# Autodesk Inventor assembly: 1420-06-00 Endstop
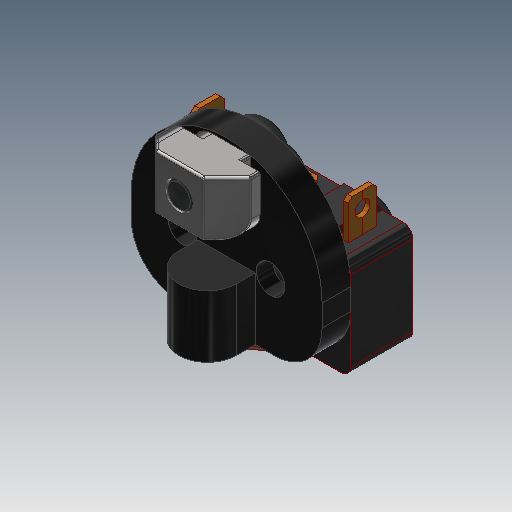
[picture p0: Inventor's stored thumbnail of the model, 512x512]
Saved by Autodesk Inventor 2017 (Build 210142000, 142)
## iProperties
Part Number: 1420-06-00 Endstop
Material: Générique
Document SubType Name: Assembly
Designer: Adrien MARY
Author: Adrien MARY
## Documents named in this file (5)
- W:\Professionnel\Conception FABLAB\1420-Vauban 3D XL\1420-06 Endstop\1420-06-00 Endstop.iam
- W:\Professionnel\Conception FABLAB\1420-Vauban 3D XL\1420-06 Endstop\1420-06-01 Support capteur.ipt
- W:\Professionnel\Conception FABLAB\1420-Vauban 3D XL\1420-06 Endstop\1420-06-02 Endstop.ipt
- W:\Professionnel\Conception FABLAB\1420-Vauban 3D XL\1420-90 Centre de contenu\fr-FR\ISO 7380-1\ISO 7380-1 - M3 x 8.ipt
- W:\Professionnel\Conception FABLAB\1420-Vauban 3D XL\1420-01 Armature\1420-01-11 Noix M3.ipt
## Components (6 placed, 4 different names)
1. 1420-06-01 Support capteur:1 — Logement:1, Placage:1, Logement:4, Affleurement:1
2. 1420-06-02 Endstop:1 — Logement:1, Placage:1, Logement:2, Logement:3
3. ISO 7380-1 M3 x 8:1 — Logement:3
4. ISO 7380-1 M3 x 8:2 — Logement:2
5. ISO 7380-1 M3 x 8:3 — Logement:4, Placage:2
6. 1420-01-11 Noix M3:1 — Affleurement:1, Placage:2
## Relationships (7: Insert 4, Mate 2, Flush 1)
- Logement:1 [Insert]: 1420-06-01 Support capteur:1 ↔ 1420-06-02 Endstop:1
- Placage:1 [Mate]: 1420-06-01 Support capteur:1 ↔ 1420-06-02 Endstop:1
- Logement:2 [Insert]: 1420-06-02 Endstop:1 ↔ ISO 7380-1 M3 x 8:2
- Logement:3 [Insert]: 1420-06-02 Endstop:1 ↔ ISO 7380-1 M3 x 8:1
- Logement:4 [Insert]: 1420-06-01 Support capteur:1 ↔ ISO 7380-1 M3 x 8:3
- Affleurement:1 [Flush] (4.5 mm): 1420-06-01 Support capteur:1 ↔ 1420-01-11 Noix M3:1
- Placage:2 [Mate]: ISO 7380-1 M3 x 8:3 ↔ 1420-01-11 Noix M3:1
